# Autodesk Inventor assembly: ASY ДМФ 0100 Барабан v2.1
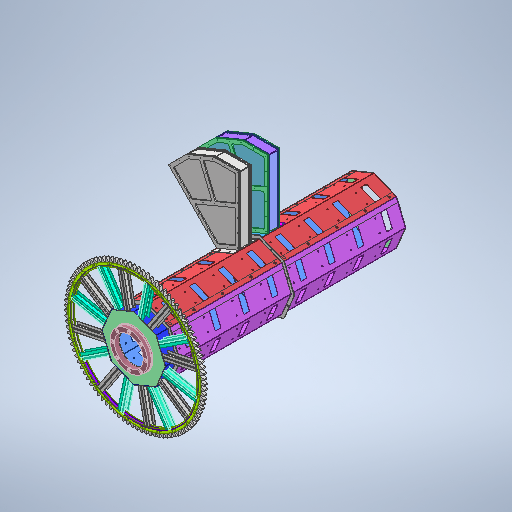
[picture p0: Inventor's stored thumbnail of the model, 512x512]
Saved by Autodesk Inventor 2025 (Build 290162010, 162A)
## iProperties
Created: 2024-04-28
Part Number: ASY ДМФ 0100 Барабан v2.1
Document SubType Name: Assembly
Designer: pokla
Author: pokla
## Documents named in this file (25)
- C:\Users\pokla\Documents\Inventor\ДФО\ДМФ\DMF-Disk-Micro-Filter\Барабан v2.1\ASY ДМФ 0100 Барабан v2.1.iam
- C:\Users\pokla\Documents\Inventor\ДФО\ДМФ\DMF-Disk-Micro-Filter\Барабан v2.1\DMF 01 21 Барабан торец НОС v2.1.ipt
- C:\Users\pokla\Documents\Inventor\ДФО\ДМФ\DMF-Disk-Micro-Filter\Барабан v2.1\DMF 01 13 Барабан Лист лев брт v2.1.ipt
- C:\Users\pokla\Documents\Inventor\ДФО\ДМФ\DMF-Disk-Micro-Filter\Барабан v2.1\DMF 01 14 Барабан Лист прав брт v2.1.ipt
- C:\Users\pokla\Documents\Inventor\ДФО\ДМФ\DMF-Disk-Micro-Filter\Барабан v2.1\DMF 01 31 Барабан Опорное кольцо НОС v2.1.ipt
- C:\Users\pokla\Documents\Inventor\ДФО\ДМФ\DMF-Disk-Micro-Filter\Барабан v2.1\DMF 01 17 опора крышки v2.1.ipt
- C:\Users\pokla\Documents\Inventor\ДФО\ДМФ\DMF-Disk-Micro-Filter\Барабан v2.1\DMF 000 размеры v2.1.ipt
- C:\Users\pokla\Documents\Inventor\ДФО\ДМФ\DMF-Disk-Micro-Filter\Барабан v2.1\DMF 01 12 Барабан усилитель v2.1.ipt
- C:\Users\pokla\Documents\Inventor\ДФО\ДМФ\DMF-Disk-Micro-Filter\Барабан v2.1\ASY DMF 010 cap v2.1.iam
- C:\Users\pokla\Documents\Inventor\ДФО\ДМФ\DMF-Disk-Micro-Filter\Барабан v2.1\DMF 01 32 Барабан Опорное кольцо КОРМА v2.1.ipt
- C:\Users\pokla\Documents\Inventor\ДФО\ДМФ\DMF-Disk-Micro-Filter\Барабан v2.1\DMF 01 22 Барабан торец КОРМА v2.1.ipt
- C:\Users\pokla\Documents\Inventor\ДФО\ДМФ\DMF-Disk-Micro-Filter\Барабан v2.1\ASY DMF filter package v2.1.iam
- C:\Users\pokla\Documents\Inventor\ДФО\ДМФ\DMF-Disk-Micro-Filter\Барабан v2.1\DMF 01 21 cylinder butt end nose.ipt
- C:\Users\pokla\Documents\Inventor\ДФО\ДМФ\DMF-Disk-Micro-Filter\Барабан v2.1\DMF 2.1 01 42 Gear way 2.ipt
- C:\Users\pokla\Documents\Inventor\ДФО\ДМФ\DMF-Disk-Micro-Filter\Барабан v2.1\DMF 2.1 01 43 Gear rim 3.ipt
- C:\Users\pokla\Documents\Inventor\ДФО\ДМФ\DMF-Disk-Micro-Filter\Барабан v2.1\DMF 2.1 01 44 Gear rim 4.ipt
- C:\Users\pokla\Documents\Inventor\ДФО\ДМФ\DMF-Disk-Micro-Filter\Барабан v2.1\DMF 2.1 01 45 Gear ring 5.ipt
- C:\Users\pokla\Documents\Inventor\ДФО\ДМФ\DMF-Disk-Micro-Filter\Барабан v2.1\DMF 2.1 01 46 Gear axis wheel 6.ipt
- C:\Users\pokla\Documents\Inventor\ДФО\ДМФ\DMF-Disk-Micro-Filter\Барабан v2.1\DMF 01 13 Барабан усилитель v2.1.ipt
- C:\Users\pokla\Documents\Inventor\ДФО\ДМФ\DMF-Disk-Micro-Filter\шестерни 06.09.2025\DMF sector big gear 2.1.ipt
- C:\Users\pokla\Documents\Inventor\ДФО\ДМФ\DMF-Disk-Micro-Filter\Барабан v2.1\DMF 01 15 drum sheet 1.ipt
- C:\Users\pokla\Documents\Inventor\ДФО\ДМФ\DMF-Disk-Micro-Filter\ДМФ 01 12 Барабан усилитель.ipt
- C:\Users\pokla\Documents\Inventor\ДФО\ДМФ\DMF-Disk-Micro-Filter\ДМФ 01 15 Барабан усилитель борта.ipt
- C:\Users\pokla\Documents\Inventor\ДФО\ДМФ\DMF-Disk-Micro-Filter\Барабан v2.1\DMF 2.1 Пластина паза маленькая.ipt
- C:\Users\pokla\Documents\Inventor\ДФО\ДМФ\DMF-Disk-Micro-Filter\Барабан v2.1\DMF 2.1 Пластина паза большая.ipt
## Components (107 placed, 36 different names)
1. DMF 000 размеры v2.1.ipt:1
2. DMF 01 21 Барабан торец НОС v2.1.ipt:1 — Mate:41, Flush:29, Flush:30, Mate:42, Flush:31, Flush:32, Rigid:80, Rigid:81
3. DMF 01 31 Барабан Опорное кольцо НОС v2.1.ipt:1 — Rigid:80
4. DMF 01 32 Барабан Опорное кольцо КОРМА v2.1.ipt:1 — Rigid:20
5. DMF 01 22 Барабан торец КОРМА v2.1.ipt:1 — Rigid:20, Rigid:51, Rigid:53, Mate:36, Flush:22, Flush:23, Mate:37, Flush:24, Flush:25, Mate:45, Flush:34, Flush:35
6. DMF 01 13 Барабан Лист лев брт v2.1.ipt:1 — Rigid:51, Rigid:69
7. DMF 01 14 Барабан Лист прав брт v2.1.ipt:1 — Rigid:53, Rigid:68
8. DMF 01 17 опора крышки v2.1.ipt:1 — Mate:37, Flush:24, Flush:25, Rigid:64
9. DMF 01 17 опора крышки v2.1.ipt:2 — Mate:36, Flush:22, Flush:23, Rigid:63
10. ASY DMF 010 cap v2.1.iam:1 [sub-assembly] — Mate:45, Flush:34, Flush:35, Flush:36, Mate:46, Mate:47, Rigid:67, Rigid:74, Rigid:75
11. DMF 01 21 cylinder butt end nose.ipt:1
12. DMF 2.1 01 45 Gear ring 5.ipt:1
13. DMF 2.1 01 46 Gear axis wheel 6.ipt:1
14. DMF 2.1 01 44 Gear rim 4.ipt:1 — Rigid:39, Rigid:40, Rigid:41
15. DMF 2.1 01 43 Gear rim 3.ipt:2 — Rigid:24, Rigid:35
16. DMF 2.1 01 43 Gear rim 3.ipt:1 — Rigid:24
17. DMF 2.1 01 43 Gear rim 3.ipt:3 — Rigid:35, Rigid:36, Rigid:39
18. DMF 2.1 01 43 Gear rim 3.ipt:4
19. DMF 2.1 01 43 Gear rim 3.ipt:5 — Rigid:36, Rigid:38, Rigid:81
20. DMF 2.1 01 43 Gear rim 3.ipt:6 — Rigid:42
21. DMF 2.1 01 43 Gear rim 3.ipt:7 — Rigid:38, Tangent:1
22. DMF 2.1 01 43 Gear rim 3.ipt:8
23. DMF 2.1 01 44 Gear rim 4.ipt:2 — Rigid:40
24. DMF 2.1 01 44 Gear rim 4.ipt:3 — Rigid:41
25. DMF 01 15 drum sheet 1.ipt:1 — Mate:41, Flush:29, Flush:30, Flush:33, Mate:43, Mate:50, Mate:51, Flush:38, Flush:39
26. DMF 01 15 drum sheet 1.ipt:2 — Mate:42, Flush:31, Flush:32, Mate:44
27. ДМФ 01 12 Барабан усилитель.ipt:1 — Rigid:54, Rigid:55, Flush:36, Mate:46, Mate:47, Rigid:70
28. ДМФ 01 15 Барабан усилитель борта.ipt:1 — Rigid:54
29. ДМФ 01 15 Барабан усилитель борта.ipt:2 — Rigid:55
30. ДМФ 01 12 Барабан усилитель.ipt:2 — Rigid:56, Rigid:57, Flush:33, Mate:43, Mate:44, Rigid:73
31. ДМФ 01 15 Барабан усилитель борта.ipt:3 — Rigid:56
32. ДМФ 01 15 Барабан усилитель борта.ipt:4 — Rigid:57
33. ASY DMF filter package v2.1.iam:1 [sub-assembly] — Rigid:59
34. DMF 2.1 01 42 Gear way 2.ipt:1 — Rigid:59, Rigid:75
35. DMF 2.1 Пластина паза маленькая.ipt:1 — Rigid:62, Rigid:74
36. DMF 2.1 Пластина паза большая:1 — Rigid:62
37. DMF 01 14 Барабан Лист прав брт v2.1:2 — Rigid:68
38. DMF 01 13 Барабан Лист лев брт v2.1:2 — Rigid:69
39. ASY DMF 010 cap v2.1:2 [sub-assembly] — Rigid:67, Flush:37, Mate:48, Mate:49, Rigid:77, Rigid:79
40. DMF 01 17 опора крышки v2.1:3 — Rigid:63
41. DMF 01 17 опора крышки v2.1:4 — Rigid:64
42. ДМФ 01 12 Барабан усилитель:3 — Rigid:70
43. ДМФ 01 15 Барабан усилитель борта:5
44. ДМФ 01 15 Барабан усилитель борта:6
45. ДМФ 01 12 Барабан усилитель:4 — Flush:37, Mate:48, Mate:49, Rigid:73
46. ДМФ 01 15 Барабан усилитель борта:7
47. ДМФ 01 15 Барабан усилитель борта:8
48. DMF 2.1 Пластина паза маленькая:2 — Rigid:77
49. DMF 2.1 Пластина паза большая:2
50. ASY DMF filter package v2.1:2 [sub-assembly]
51. DMF 2.1 01 42 Gear way 2:2 — Rigid:79
52. DMF sector big gear 2.1.ipt:1 — Rigid:42
53. DMF sector big gear 2.1:2
54. DMF sector big gear 2.1:3
55. DMF sector big gear 2.1:4
56. DMF sector big gear 2.1:5
57. DMF sector big gear 2.1:6
58. DMF sector big gear 2.1:7
59. DMF sector big gear 2.1:8
60. DMF sector big gear 2.1:9
61. DMF sector big gear 2.1:10
62. DMF sector big gear 2.1:11
63. DMF sector big gear 2.1:12
64. DMF sector big gear 2.1:13
65. DMF sector big gear 2.1:14
66. DMF sector big gear 2.1:15
67. DMF sector big gear 2.1:16
68. DMF sector big gear 2.1:17
69. DMF sector big gear 2.1:18
70. DMF sector big gear 2.1:19
71. DMF sector big gear 2.1:20
72. DMF sector big gear 2.1:21
73. DMF sector big gear 2.1:22
74. DMF sector big gear 2.1:23
75. DMF sector big gear 2.1:24
76. DMF 01 12 Барабан усилитель v2.1.ipt:1 — Rigid:82, Symmetry:1, Mate:51, Flush:39
77. DMF 01 13 Барабан усилитель v2.1.ipt:1 — Rigid:82
78. DMF 01 12 Барабан усилитель v2.1.ipt:2 — Rigid:83, Symmetry:1, Mate:50, Flush:38
79. DMF 01 13 Барабан усилитель v2.1.ipt:2 — Rigid:83, Tangent:1
80. DMF 01 12 Барабан усилитель v2.1:52
81. ДМФ 01 13 Барабан усилитель v2.0:3
82. DMF 01 12 Барабан усилитель v2.1:53
83. ДМФ 01 13 Барабан усилитель v2.0:4
84. DMF 01 12 Барабан усилитель v2.1:54
85. ДМФ 01 13 Барабан усилитель v2.0:5
86. DMF 01 12 Барабан усилитель v2.1:55
87. ДМФ 01 13 Барабан усилитель v2.0:6
88. DMF 01 12 Барабан усилитель v2.1:56
89. ДМФ 01 13 Барабан усилитель v2.0:7
90. DMF 01 12 Барабан усилитель v2.1:57
91. ДМФ 01 13 Барабан усилитель v2.0:8
92. DMF 01 12 Барабан усилитель v2.1:58
93. ДМФ 01 13 Барабан усилитель v2.0:9
94. DMF 01 12 Барабан усилитель v2.1:59
95. ДМФ 01 13 Барабан усилитель v2.0:10
96. DMF 01 12 Барабан усилитель v2.1:60
97. ДМФ 01 13 Барабан усилитель v2.0:11
98. DMF 01 12 Барабан усилитель v2.1:61
99. ДМФ 01 13 Барабан усилитель v2.0:12
100. DMF 01 12 Барабан усилитель v2.1:62
101. ДМФ 01 13 Барабан усилитель v2.0:13
102. DMF 01 12 Барабан усилитель v2.1:63
103. ДМФ 01 13 Барабан усилитель v2.0:14
104. DMF 01 12 Барабан усилитель v2.1:64
105. ДМФ 01 13 Барабан усилитель v2.0:15
106. DMF 01 12 Барабан усилитель v2.1:65
107. ДМФ 01 13 Барабан усилитель v2.0:16
## Component patterns: (24 elements, first: DMF sector big gear 2.1.ipt:1), (8 elements, first: DMF 01 12 Барабан усилитель v2.1.ipt:1 + DMF 01 13 Барабан усилитель v2.1.ipt:1 + DMF 01 12 Барабан усилитель v2.1.ipt:2 + DMF 01 13 Барабан усилитель v2.1.ipt:2)
## Relationships (71: WeldJoint 41, Flush 15, Mate 13, Symmetry 1, Tangent 1)
- Rigid:20 [WeldJoint]: DMF 01 32 Барабан Опорное кольцо КОРМА v2.1.ipt:1 ↔ DMF 01 22 Барабан торец КОРМА v2.1.ipt:1
- Rigid:24 [WeldJoint] (25 mm): DMF 2.1 01 43 Gear rim 3.ipt:2 ↔ DMF 2.1 01 43 Gear rim 3.ipt:1
- [WeldJoint] (25 mm): DMF 2.1 01 43 Gear rim 3.ipt:3 ↔ DMF 2.1 01 43 Gear rim 3.ipt:4
- [WeldJoint] (25 mm): DMF 2.1 01 43 Gear rim 3.ipt:5 ↔ DMF 2.1 01 43 Gear rim 3.ipt:6
- Rigid:35 [WeldJoint]: DMF 2.1 01 43 Gear rim 3.ipt:2 ↔ DMF 2.1 01 43 Gear rim 3.ipt:3
- Rigid:36 [WeldJoint]: DMF 2.1 01 43 Gear rim 3.ipt:3 ↔ DMF 2.1 01 43 Gear rim 3.ipt:5
- [WeldJoint] (25 mm): DMF 2.1 01 43 Gear rim 3.ipt:7 ↔ DMF 2.1 01 43 Gear rim 3.ipt:8
- Rigid:38 [WeldJoint]: DMF 2.1 01 43 Gear rim 3.ipt:5 ↔ DMF 2.1 01 43 Gear rim 3.ipt:7
- Rigid:39 [WeldJoint]: DMF 2.1 01 44 Gear rim 4.ipt:1 ↔ DMF 2.1 01 43 Gear rim 3.ipt:3
- Rigid:40 [WeldJoint]: DMF 2.1 01 44 Gear rim 4.ipt:1 ↔ DMF 2.1 01 44 Gear rim 4.ipt:2
- Rigid:41 [WeldJoint]: DMF 2.1 01 44 Gear rim 4.ipt:1 ↔ DMF 2.1 01 44 Gear rim 4.ipt:3
- Rigid:42 [WeldJoint]: DMF 2.1 01 43 Gear rim 3.ipt:6 ↔ DMF sector big gear 2.1.ipt:1
- Rigid:51 [WeldJoint]: DMF 01 22 Барабан торец КОРМА v2.1.ipt:1 ↔ DMF 01 13 Барабан Лист лев брт v2.1.ipt:1
- Rigid:53 [WeldJoint]: DMF 01 22 Барабан торец КОРМА v2.1.ipt:1 ↔ DMF 01 14 Барабан Лист прав брт v2.1.ipt:1
- Mate:36: DMF 01 22 Барабан торец КОРМА v2.1.ipt:1 ↔ DMF 01 17 опора крышки v2.1.ipt:2
- Flush:22 (2 mm): DMF 01 22 Барабан торец КОРМА v2.1.ipt:1 ↔ DMF 01 17 опора крышки v2.1.ipt:2
- Flush:23 (2 mm): DMF 01 22 Барабан торец КОРМА v2.1.ipt:1 ↔ DMF 01 17 опора крышки v2.1.ipt:2
- Mate:37: DMF 01 22 Барабан торец КОРМА v2.1.ipt:1 ↔ DMF 01 17 опора крышки v2.1.ipt:1
- Flush:24 (2 mm): DMF 01 22 Барабан торец КОРМА v2.1.ipt:1 ↔ DMF 01 17 опора крышки v2.1.ipt:1
- Flush:25 (2 mm): DMF 01 22 Барабан торец КОРМА v2.1.ipt:1 ↔ DMF 01 17 опора крышки v2.1.ipt:1
- Rigid:54 [WeldJoint]: ДМФ 01 12 Барабан усилитель.ipt:1 ↔ ДМФ 01 15 Барабан усилитель борта.ipt:1
- Rigid:55 [WeldJoint]: ДМФ 01 12 Барабан усилитель.ipt:1 ↔ ДМФ 01 15 Барабан усилитель борта.ipt:2
- Rigid:56 [WeldJoint]: ДМФ 01 12 Барабан усилитель.ipt:2 ↔ ДМФ 01 15 Барабан усилитель борта.ipt:3
- Rigid:57 [WeldJoint]: ДМФ 01 12 Барабан усилитель.ipt:2 ↔ ДМФ 01 15 Барабан усилитель борта.ipt:4
- Mate:41: DMF 01 21 Барабан торец НОС v2.1.ipt:1 ↔ DMF 01 15 drum sheet 1.ipt:1
- Flush:29: DMF 01 21 Барабан торец НОС v2.1.ipt:1 ↔ DMF 01 15 drum sheet 1.ipt:1
- Flush:30: DMF 01 21 Барабан торец НОС v2.1.ipt:1 ↔ DMF 01 15 drum sheet 1.ipt:1
- Mate:42: DMF 01 21 Барабан торец НОС v2.1.ipt:1 ↔ DMF 01 15 drum sheet 1.ipt:2
- Flush:31: DMF 01 21 Барабан торец НОС v2.1.ipt:1 ↔ DMF 01 15 drum sheet 1.ipt:2
- Flush:32: DMF 01 21 Барабан торец НОС v2.1.ipt:1 ↔ DMF 01 15 drum sheet 1.ipt:2
- Flush:33: DMF 01 15 drum sheet 1.ipt:1 ↔ ДМФ 01 12 Барабан усилитель.ipt:2
- Mate:43: DMF 01 15 drum sheet 1.ipt:1 ↔ ДМФ 01 12 Барабан усилитель.ipt:2
- Mate:44: DMF 01 15 drum sheet 1.ipt:2 ↔ ДМФ 01 12 Барабан усилитель.ipt:2
- Mate:45: DMF 01 22 Барабан торец КОРМА v2.1.ipt:1 ↔ ASY DMF 010 cap v2.1.iam:1
- Flush:34: DMF 01 22 Барабан торец КОРМА v2.1.ipt:1 ↔ ASY DMF 010 cap v2.1.iam:1
- Flush:35: DMF 01 22 Барабан торец КОРМА v2.1.ipt:1 ↔ ASY DMF 010 cap v2.1.iam:1
- Flush:36: ASY DMF 010 cap v2.1.iam:1 ↔ ДМФ 01 12 Барабан усилитель.ipt:1
- Mate:46: ASY DMF 010 cap v2.1.iam:1 ↔ ДМФ 01 12 Барабан усилитель.ipt:1
- Mate:47: ASY DMF 010 cap v2.1.iam:1 ↔ ДМФ 01 12 Барабан усилитель.ipt:1
- Rigid:59 [WeldJoint] (5 mm): ASY DMF filter package v2.1.iam:1 ↔ DMF 2.1 01 42 Gear way 2.ipt:1
- Rigid:62 [WeldJoint]: DMF 2.1 Пластина паза маленькая.ipt:1 ↔ DMF 2.1 Пластина паза большая:1
- Rigid:63 [WeldJoint]: DMF 01 17 опора крышки v2.1.ipt:2 ↔ DMF 01 17 опора крышки v2.1:3
- Rigid:64 [WeldJoint]: DMF 01 17 опора крышки v2.1.ipt:1 ↔ DMF 01 17 опора крышки v2.1:4
- [WeldJoint]: ДМФ 01 12 Барабан усилитель:3 ↔ ДМФ 01 15 Барабан усилитель борта:5
- [WeldJoint]: ДМФ 01 12 Барабан усилитель:3 ↔ ДМФ 01 15 Барабан усилитель борта:6
- Rigid:67 [WeldJoint]: ASY DMF 010 cap v2.1.iam:1 ↔ ASY DMF 010 cap v2.1:2
- Rigid:68 [WeldJoint]: DMF 01 14 Барабан Лист прав брт v2.1.ipt:1 ↔ DMF 01 14 Барабан Лист прав брт v2.1:2
- Rigid:69 [WeldJoint]: DMF 01 13 Барабан Лист лев брт v2.1.ipt:1 ↔ DMF 01 13 Барабан Лист лев брт v2.1:2
- Rigid:70 [WeldJoint]: ДМФ 01 12 Барабан усилитель.ipt:1 ↔ ДМФ 01 12 Барабан усилитель:3
- [WeldJoint]: ДМФ 01 12 Барабан усилитель:4 ↔ ДМФ 01 15 Барабан усилитель борта:7
- [WeldJoint]: ДМФ 01 12 Барабан усилитель:4 ↔ ДМФ 01 15 Барабан усилитель борта:8
- Flush:37: ASY DMF 010 cap v2.1:2 ↔ ДМФ 01 12 Барабан усилитель:4
- Mate:48: ASY DMF 010 cap v2.1:2 ↔ ДМФ 01 12 Барабан усилитель:4
- Mate:49: ASY DMF 010 cap v2.1:2 ↔ ДМФ 01 12 Барабан усилитель:4
- Rigid:73 [WeldJoint]: ДМФ 01 12 Барабан усилитель.ipt:2 ↔ ДМФ 01 12 Барабан усилитель:4
- Rigid:74 [WeldJoint] (-48.5 mm): ASY DMF 010 cap v2.1.iam:1 ↔ DMF 2.1 Пластина паза маленькая.ipt:1
- Rigid:75 [WeldJoint]: ASY DMF 010 cap v2.1.iam:1 ↔ DMF 2.1 01 42 Gear way 2.ipt:1
- [WeldJoint]: DMF 2.1 Пластина паза маленькая:2 ↔ DMF 2.1 Пластина паза большая:2
- Rigid:77 [WeldJoint] (-48.5 mm): ASY DMF 010 cap v2.1:2 ↔ DMF 2.1 Пластина паза маленькая:2
- [WeldJoint] (5 mm): ASY DMF filter package v2.1:2 ↔ DMF 2.1 01 42 Gear way 2:2
- Rigid:79 [WeldJoint]: ASY DMF 010 cap v2.1:2 ↔ DMF 2.1 01 42 Gear way 2:2
- Rigid:80 [WeldJoint]: DMF 01 21 Барабан торец НОС v2.1.ipt:1 ↔ DMF 01 31 Барабан Опорное кольцо НОС v2.1.ipt:1
- Rigid:81 [WeldJoint] (-5 mm): DMF 01 21 Барабан торец НОС v2.1.ipt:1 ↔ DMF 2.1 01 43 Gear rim 3.ipt:5
- Rigid:82 [WeldJoint]: DMF 01 12 Барабан усилитель v2.1.ipt:1 ↔ DMF 01 13 Барабан усилитель v2.1.ipt:1
- Rigid:83 [WeldJoint]: DMF 01 12 Барабан усилитель v2.1.ipt:2 ↔ DMF 01 13 Барабан усилитель v2.1.ipt:2
- Symmetry:1: DMF 01 12 Барабан усилитель v2.1.ipt:1 ↔ DMF 01 12 Барабан усилитель v2.1.ipt:2
- Mate:50: DMF 01 15 drum sheet 1.ipt:1 ↔ DMF 01 12 Барабан усилитель v2.1.ipt:2
- Mate:51: DMF 01 15 drum sheet 1.ipt:1 ↔ DMF 01 12 Барабан усилитель v2.1.ipt:1
- Flush:38: DMF 01 15 drum sheet 1.ipt:1 ↔ DMF 01 12 Барабан усилитель v2.1.ipt:2
- Flush:39: DMF 01 15 drum sheet 1.ipt:1 ↔ DMF 01 12 Барабан усилитель v2.1.ipt:1
- Tangent:1: DMF 2.1 01 43 Gear rim 3.ipt:7 ↔ DMF 01 13 Барабан усилитель v2.1.ipt:2
## Named parameters: d314_d251 = 25 mm, d315_d251 = 25 mm, d318_d251 = 25 mm, d414_d373 = 0 mm, d415_d374 = 0 mm, d420_d373 = 0 mm, d421_d374 = 0 mm, d428_d406 = 0 mm, d430_d399 = 5 mm
